# Autodesk Inventor assembly: Montagem
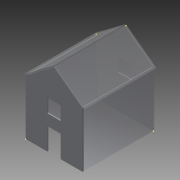
[picture p0: Inventor's stored thumbnail of the model, 180x180]
Saved by Autodesk Inventor 2015 (Build 190159000, 159)
## iProperties
Created: 2016-08-07
Part Number: Montagem
Document SubType Name: Assembly
Designer: Gabriel
Author: Gabriel
## Documents named in this file (5)
- C:\Users\Gabriel\Desktop\TCC\Montagem.iam
- C:\Users\Gabriel\Desktop\TCC\frente.ipt
- C:\Users\Gabriel\Desktop\TCC\fundo.ipt
- C:\Users\Gabriel\Desktop\TCC\lateral.ipt
- C:\Users\Gabriel\Desktop\TCC\teto01.ipt
## Components (6 placed, 4 different names)
1. frente:1 — Rotational:1, Rotational:2, Rotational:9, Rotational:10
2. fundo:1 — Rotational:3, Rotational:4, Planar:1, Rotational:7, Rotational:8
3. lateral:1 — Rotational:2, Rotational:4
4. lateral:2 — Rotational:1, Rotational:3, Planar:1
5. teto01:1 — Rotational:8, Rotational:9
6. teto01:2 — Rotational:7, Rotational:10
## Relationships (9: RevoluteJoint 8, PlanarJoint 1)
- Rotational:1 [RevoluteJoint]: frente:1 ↔ lateral:2
- Rotational:2 [RevoluteJoint]: frente:1 ↔ lateral:1
- Rotational:3 [RevoluteJoint]: fundo:1 ↔ lateral:2
- Rotational:4 [RevoluteJoint]: fundo:1 ↔ lateral:1
- Planar:1: fundo:1 ↔ lateral:2
- Rotational:7 [RevoluteJoint]: fundo:1 ↔ teto01:2
- Rotational:8 [RevoluteJoint]: fundo:1 ↔ teto01:1
- Rotational:9 [RevoluteJoint]: frente:1 ↔ teto01:1
- Rotational:10 [RevoluteJoint]: frente:1 ↔ teto01:2
